# Autodesk Inventor assembly: Assembly 2.0
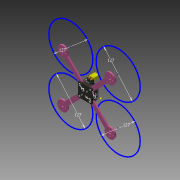
[picture p0: Inventor's stored thumbnail of the model, 180x180]
Saved by Autodesk Inventor 2015 (Build 190159000, 159)
## iProperties
Created: 2017-01-15
Part Number: Assembly 2.0
Document SubType Name: Assembly
Designer: Per
Author: Per
## Documents named in this file (8)
- C:\Users\Per\Desktop\Prototyp X Quad\Version 2.0\Assembly 2.0.iam
- C:\Users\Per\Desktop\Prototyp X Quad\Version 2.0\Bot.ipt
- C:\Users\Per\Desktop\Prototyp X Quad\Version 2.0\Arm2.ipt
- C:\Users\Per\Desktop\Prototyp X Quad\Version 2.0\Topp.ipt
- C:\Users\Per\Desktop\Prototyp X Quad\Version 2.0\M3x13.ipt
- C:\Users\Per\Desktop\Prototyp X Quad\Version 2.0\Standoff.ipt
- C:\Users\Per\Desktop\Prototyp X Quad\Version 2.0\HGLRC PDB.iam
- C:\Users\Per\Desktop\Prototyp X Quad\Version 2.0\Naze32 Acro.ipt
## Components (24 placed, 7 different names)
1. Bot:1 — Rigid:1, Cylindrical:1, Cylindrical:2, Cylindrical:3, Rigid:2, Insert:5, Insert:6, Insert:7, Insert:8
2. Arm2:1 — Cylindrical:3
3. Arm2:2 — Cylindrical:2
4. Arm2:3 — Cylindrical:1
5. Arm2:4 — Rigid:1
6. Topp:1 — Rigid:2, Insert:1, Insert:2, Insert:3, Insert:4, Insert:9, Insert:10, Insert:11, Insert:12
7. M3x13:1 — Insert:2
8. M3x13:2 — Insert:3
9. M3x13:3 — Insert:4
10. M3x13:4 — Insert:5
11. M3x13:5 — Insert:6
12. M3x13:6 — Insert:7
13. M3x13:7 — Insert:8
14. M3x13:8 — Insert:1
15. Standoff:1 — Insert:11
16. Standoff:2 — Insert:12
17. Standoff:3 — Insert:10
18. Standoff:4 — Insert:9, Insert:13
19. HGLRC PDB:1 [sub-assembly] — Insert:13, Insert:14, Insert:15, Insert:16, Insert:17
20. Standoff:5 — Insert:15
21. Standoff:6 — Insert:14
22. Standoff:7 — Insert:16
23. Standoff:8 — Insert:17, Insert:18
24. Naze32 Acro:1 — Insert:18
## Relationships (23: Insert 18, CylindricalJoint 3, WeldJoint 2)
- Rigid:1 [WeldJoint]: Bot:1 ↔ Arm2:4
- Cylindrical:1: Bot:1 ↔ Arm2:3
- Cylindrical:2: Bot:1 ↔ Arm2:2
- Cylindrical:3: Bot:1 ↔ Arm2:1
- Rigid:2 [WeldJoint]: Bot:1 ↔ Topp:1
- Insert:1: Topp:1 ↔ M3x13:8
- Insert:2: Topp:1 ↔ M3x13:1
- Insert:3: Topp:1 ↔ M3x13:2
- Insert:4: Topp:1 ↔ M3x13:3
- Insert:5: Bot:1 ↔ M3x13:4
- Insert:6: Bot:1 ↔ M3x13:5
- Insert:7: Bot:1 ↔ M3x13:6
- Insert:8: Bot:1 ↔ M3x13:7
- Insert:9: Topp:1 ↔ Standoff:4
- Insert:10: Topp:1 ↔ Standoff:3
- Insert:11: Topp:1 ↔ Standoff:1
- Insert:12: Topp:1 ↔ Standoff:2
- Insert:13: Standoff:4 ↔ HGLRC PDB:1
- Insert:14: HGLRC PDB:1 ↔ Standoff:6
- Insert:15: HGLRC PDB:1 ↔ Standoff:5
- Insert:16: HGLRC PDB:1 ↔ Standoff:7
- Insert:17: HGLRC PDB:1 ↔ Standoff:8
- Insert:18: Standoff:8 ↔ Naze32 Acro:1
